# Autodesk Inventor assembly: Inner
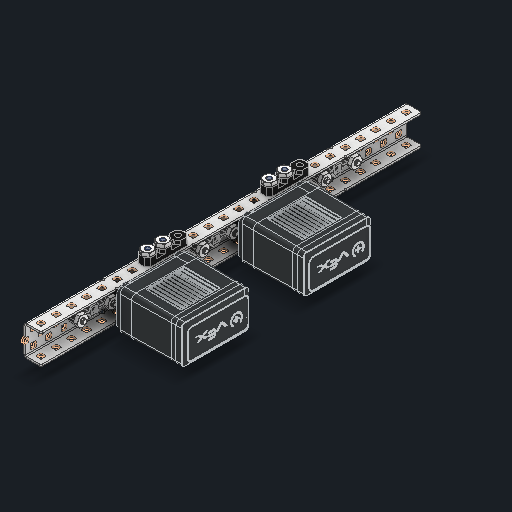
[picture p0: Inventor's stored thumbnail of the model, 512x512]
Saved by Autodesk Inventor 2025.1 (Build 291241000, 241)
## iProperties
Created: 2024-11-28
Part Number: Inner
Document SubType Name: Assembly
Designer: avere
Author: avere
## Documents named in this file (12)
- C:\Users\avere\VEX\High Stakes\CAD\Codie\Chassis\Drivebay Left\Inner\Inner.iam
- C:\Users\avere\VEX\High Stakes\CAD\Codie\Chassis\Drivebay Left\Inner\Alu C 1x2x1x25.ipt
- C:\Users\avere\VEX\High Stakes\CAD\Codie\Chassis\Drivebay Left\Inner\Gear Layout.ipt
- C:\Users\avere\VEX\High Stakes\CAD\Codie\Chassis\Drivebay Left\Inner\Bearing Flat NScrew Slotted.iam
- C:\Users\avere\VEX\High Stakes\CAD\Codie\Chassis\Drivebay Left\Inner\Nut Keps.ipt
- C:\Users\avere\VEX\High Stakes\CAD\Codie\Chassis\Drivebay Left\Inner\Bearing Flat.ipt
- C:\Users\avere\VEX\High Stakes\CAD\ROBOPROS-CAD-Inventor\Structure\Hardware\Nut Nylon\Nut Nylon - White.ipt
- C:\Users\avere\VEX\High Stakes\CAD\ROBOPROS-CAD-Inventor\Structure\Hardware\Nut Nylon.ipt
- C:\Users\avere\VEX\High Stakes\CAD\ROBOPROS-CAD-Inventor\Structure\Hardware\Screw Steel - Star\SScrew Star Smooth 1.750.ipt
- C:\Users\avere\VEX\High Stakes\CAD\ROBOPROS-CAD-Inventor\Structure\Hardware\Screw Steel - Star.ipt
- C:\Users\avere\VEX\High Stakes\CAD\ROBOPROS-CAD-Inventor\Electronics\Motors with Screws\SteelM-StarS.iam
- C:\Users\avere\VEX\High Stakes\CAD\ROBOPROS-CAD-Inventor\Electronics\Motors with Screws.iam
## Components (25 placed, 8 different names)
1. Alu C 1x2x1x25:1 — Mate:1, Flush:2, Flush:1, Mate:5, Mate:4, Mate:6, Insert:1, Insert:7, Insert:6, Insert:5, Insert:4, Mate:7, Insert:8, Insert:12, Insert:11, Insert:11, Mate:7, Insert:12, Mate:8
2. Gear Layout:1 — Mate:5, Mate:4
3. SteelM-StarS:1 [sub-assembly] — Insert:12, Mate:8
4. SteelM-StarS:2 [sub-assembly] — Insert:11, Mate:7
5. Nut Keps:1 — Insert:7
6. Nut Keps:2 — Insert:6
7. Nut Keps:3 — Insert:5
8. Nut Keps:4 — Insert:4
9. Bearing Flat:1 — Mate:7, Insert:8, Insert:10, Insert:9
10. Nut Nylon - White:1 — Insert:10
11. Nut Nylon - White:2 — Insert:9
12. SScrew Star Smooth 1.750:1 — Insert:12
13. SScrew Star Smooth 1.750:2 — Insert:11
14. Nut Keps:5
15. Nut Keps:6
16. Nut Keps:7
17. Nut Keps:8
18. Bearing Flat:2
19. Nut Nylon - White:3
20. Nut Nylon - White:4
21. SScrew Star Smooth 1.750:3
22. SScrew Star Smooth 1.750:4
23. Bearing Flat NScrew Slotted:1 [sub-assembly] — Mate:6, Insert:1
24. Bearing Flat NScrew Slotted:2 [sub-assembly]
25. Bearing Flat NScrew Slotted:3 [sub-assembly]
## Component patterns: (2 elements, first: Nut Keps:1 + Nut Keps:2 + Nut Keps:3 + Nut Keps:4 + Bearing Flat:1 + Nut Nylon - White:1 + Nut Nylon - White:2 + SScrew Star Smooth 1.750:1 + SScrew Star Smooth 1.750:2), (3 elements, first: Bearing Flat NScrew Slotted:1)
## Relationships (21: Insert 12, Mate 8, Flush 1)
- Mate:1: Alu C 1x2x1x25:1
- Flush:2 (-12.7 mm): Alu C 1x2x1x25:1
- Flush:1 [Mate] (-158.75 mm): Alu C 1x2x1x25:1
- Mate:5: Alu C 1x2x1x25:1 ↔ Gear Layout:1
- Mate:4: Alu C 1x2x1x25:1 ↔ Gear Layout:1
- Mate:6: Alu C 1x2x1x25:1 ↔ Bearing Flat NScrew Slotted:1
- Insert:1: Alu C 1x2x1x25:1 ↔ Bearing Flat NScrew Slotted:1
- Insert:7: Alu C 1x2x1x25:1 ↔ Nut Keps:1
- Insert:6: Alu C 1x2x1x25:1 ↔ Nut Keps:2
- Insert:5: Alu C 1x2x1x25:1 ↔ Nut Keps:3
- Insert:4: Alu C 1x2x1x25:1 ↔ Nut Keps:4
- Mate:7: Alu C 1x2x1x25:1 ↔ Bearing Flat:1
- Insert:8: Alu C 1x2x1x25:1 ↔ Bearing Flat:1
- Insert:10: Bearing Flat:1 ↔ Nut Nylon - White:1
- Insert:9: Bearing Flat:1 ↔ Nut Nylon - White:2
- Insert:12 (9.525 mm): Alu C 1x2x1x25:1 ↔ SScrew Star Smooth 1.750:1
- Insert:11 (9.525 mm): Alu C 1x2x1x25:1 ↔ SScrew Star Smooth 1.750:2
- Insert:11: Alu C 1x2x1x25:1 ↔ SteelM-StarS:2
- Mate:7: Alu C 1x2x1x25:1 ↔ SteelM-StarS:2
- Insert:12: Alu C 1x2x1x25:1 ↔ SteelM-StarS:1
- Mate:8: Alu C 1x2x1x25:1 ↔ SteelM-StarS:1
